# Autodesk Inventor assembly: (FINAL) Extention and 20 Degree Body Assembly
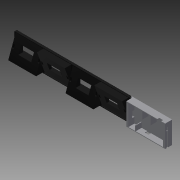
[picture p0: Inventor's stored thumbnail of the model, 180x180]
Saved by Autodesk Inventor 2017 (Build 210142000, 142)
## iProperties
Created: 2018-11-26
Part Number: (FINAL) Extention and 20 Degree Body Assembly
Document SubType Name: Assembly
Designer: eszcz
Author: eszcz
## Documents named in this file (3)
- C:\Users\eszcz\Documents\Clemson University\Ph.D Research\Nicole\Waldo Parts Inventor Parts\(FINAL) Extention and 20 Degree Body Assembly.iam
- C:\Users\eszcz\Documents\Clemson University\Ph.D Research\Nicole\Waldo Parts Inventor Parts\Waldo Extention.ipt
- C:\Users\eszcz\Documents\Clemson University\Ph.D Research\Nicole\Waldo Parts Inventor Parts\Waldo Full Body at 20 degrees.ipt
## Components (2 placed, 2 different names)
1. Waldo Full Body at 20 degrees:1 — Mate:1, Flush:1, Flush:2
2. Waldo Extention:1 — Mate:1, Flush:1, Flush:2
## Relationships (3: Flush 2, Mate 1)
- Mate:1: Waldo Full Body at 20 degrees:1 ↔ Waldo Extention:1
- Flush:1: Waldo Full Body at 20 degrees:1 ↔ Waldo Extention:1
- Flush:2: Waldo Full Body at 20 degrees:1 ↔ Waldo Extention:1
